# Autodesk Inventor assembly: Plateau
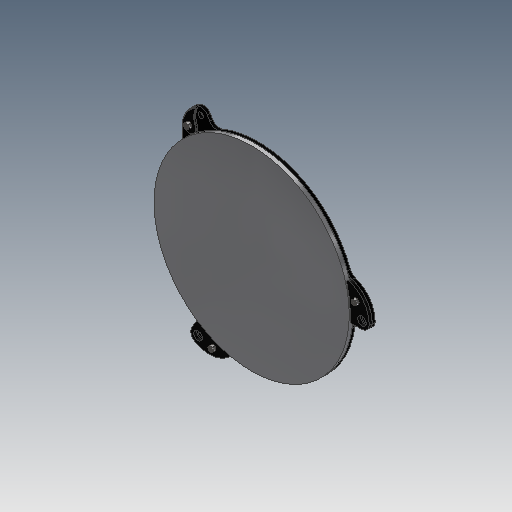
[picture p0: Inventor's stored thumbnail of the model, 512x512]
Saved by Autodesk Inventor 2017 (Build 210142000, 142)
## iProperties
Company: FABLAB Frenchmakers
Part Number: Plateau
Material: Générique
Document SubType Name: Assembly
Designer: FABLAB Frenchmakers
Project: 1420 Vauban 3D XL
Catalog Web Link: http://frenchmakers.com/
Stock Number: 1420-04-00
## Documents named in this file (8)
- W:\Professionnel\Conception FABLAB\1420-Vauban 3D XL\1420-04 Plateau\1420-04-00 Plateau.iam
- W:\Professionnel\Conception FABLAB\1420-Vauban 3D XL\1420-04 Plateau\1420-04-01 Plateau metalique.ipt
- W:\Professionnel\Conception FABLAB\1420-Vauban 3D XL\1420-04 Plateau\1420-04-04 Bloque plateau.ipt
- W:\Professionnel\Conception FABLAB\1420-Vauban 3D XL\1420-04 Plateau\1420-04-03 Plateau verre D200.ipt
- W:\Professionnel\Conception FABLAB\1420-Vauban 3D XL\1420-90 Centre de contenu\fr-FR\ANSI B18.3.1M(1)\ANSI B18.3.1M - M3x0,5 x 6(2).ipt
- W:\Professionnel\Conception FABLAB\1420-Vauban 3D XL\1420-04 Plateau\1420-04-04 Came.ipt
- W:\Professionnel\Conception FABLAB\1420-Vauban 3D XL\1420-90 Centre de contenu\fr-FR\ANSI B18.3.1M(1)\ANSI B18.3.1M - M3x0,5 x 8(2).ipt
- W:\Professionnel\Conception FABLAB\1420-Vauban 3D XL\1420-90 Centre de contenu\fr-FR\DIN 985\DIN 985 - M3.ipt
## Components (9 placed, 7 different names)
1. 1420-04-01 Plateau metalique:1 — Placage:7, Placage:10, Placage:11, Placage:12, Placage:15, Logement:1, Placage:16, Logement:3, Placage:18
2. 1420-04-04 Bloque plateau:3 — Logement:3, Placage:17
3. 1420-04-04 Bloque plateau:4 — Logement:1, Logement:2
4. 1420-04-03 Plateau verre D200:1 — Placage:7, Placage:8
5. Vis à tête percée - Métrique M3x0,5 x 6:1 — Affleurement:2, Logement:2, Placage:16
6. Vis à tête percée - Métrique M3x0,5 x 6:2 — Affleurement:2, Placage:17, Placage:18
7. Vis à tête percée - Métrique M3x0,5 x 8:1 — Placage:10, Affleurement:14, Placage:14
8. 1420-04-04 Came:1 — Placage:11, Placage:12, Affleurement:14
9. DIN 985 - Remplacé par DIN EN ISO 10511 M3:1 — Placage:14, Placage:15
## Relationships (15: Mate 10, Insert 3, Flush 2)
- Placage:7 [Mate]: 1420-04-01 Plateau metalique:1 ↔ 1420-04-03 Plateau verre D200:1
- Placage:8 [Mate]: 1420-04-03 Plateau verre D200:1
- Affleurement:2 [Flush]: Vis à tête percée - Métrique M3x0,5 x 6:1 ↔ Vis à tête percée - Métrique M3x0,5 x 6:2
- Placage:10 [Mate]: 1420-04-01 Plateau metalique:1 ↔ Vis à tête percée - Métrique M3x0,5 x 8:1
- Placage:11 [Mate]: 1420-04-01 Plateau metalique:1 ↔ 1420-04-04 Came:1
- Placage:12 [Mate]: 1420-04-01 Plateau metalique:1 ↔ 1420-04-04 Came:1
- Affleurement:14 [Flush]: Vis à tête percée - Métrique M3x0,5 x 8:1 ↔ 1420-04-04 Came:1
- Placage:14 [Mate]: Vis à tête percée - Métrique M3x0,5 x 8:1 ↔ DIN 985 - Remplacé par DIN EN ISO 10511 M3:1
- Placage:15 [Mate]: 1420-04-01 Plateau metalique:1 ↔ DIN 985 - Remplacé par DIN EN ISO 10511 M3:1
- Logement:1 [Insert]: 1420-04-01 Plateau metalique:1 ↔ 1420-04-04 Bloque plateau:4
- Logement:2 [Insert]: 1420-04-04 Bloque plateau:4 ↔ Vis à tête percée - Métrique M3x0,5 x 6:1
- Placage:16 [Mate]: 1420-04-01 Plateau metalique:1 ↔ Vis à tête percée - Métrique M3x0,5 x 6:1
- Logement:3 [Insert]: 1420-04-01 Plateau metalique:1 ↔ 1420-04-04 Bloque plateau:3
- Placage:17 [Mate]: 1420-04-04 Bloque plateau:3 ↔ Vis à tête percée - Métrique M3x0,5 x 6:2
- Placage:18 [Mate]: 1420-04-01 Plateau metalique:1 ↔ Vis à tête percée - Métrique M3x0,5 x 6:2
